# Autodesk Inventor assembly: 6 Axis Manipulator Assembly
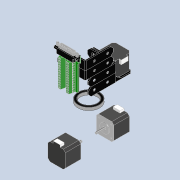
[picture p0: Inventor's stored thumbnail of the model, 180x180]
Saved by Autodesk Inventor 2022 (Build 260153000, 153)
## iProperties
Created: 2021-12-24
Part Number: 6 Axis Manipulator Assembly
Document SubType Name: Assembly
Designer: Coy
Author: Coy
## Documents named in this file (6)
- H:\3D Files\Project 3D Models\Breakfast Maker 2000\Assemblys\6 Axis Manipulator Assembly.iam
- H:\3D Files\Project 3D Models\Breakfast Maker 2000\Motors\Nema 17 Stepper Motor 37mm.ipt
- H:\3D Files\Project 3D Models\Breakfast Maker 2000\90 deg Shelf 4 Hole Bracket.ipt
- H:\3D Files\Project 3D Models\Breakfast Maker 2000\Bearings\40mm ID 52mm OD 7mm Deep Roller Bearing (2021_08_15 23_37_01 UTC).ipt
- H:\3D Files\Project 3D Models\Breakfast Maker 2000\25Pin D SUB Male Connector.ipt
- H:\3D Files\Project 3D Models\Breakfast Maker 2000\Nema 17 Stepper Motor Mounting Bracket.ipt
## Components (10 placed, 5 different names)
1. Nema 17 Stepper Motor 37mm:1
2. Nema 17 Stepper Motor 37mm:2
3. Nema 17 Stepper Motor 37mm:3 — Mate:5, Mate:6, Angle:1
4. 90 deg Shelf 4 Hole Bracket:1 — Mate:1, Flush:1, Flush:2
5. 90 deg Shelf 4 Hole Bracket:2 — Mate:1, Flush:1, Flush:2, Flush:3, Mate:3, Flush:6
6. 90 deg Shelf 4 Hole Bracket:3 — Flush:3, Flush:4, Mate:2, Flush:5, Mate:3, Flush:6, Flush:7, Flush:8
7. 90 deg Shelf 4 Hole Bracket:4 — Flush:4, Mate:2, Flush:5, Mate:4
8. 40mm ID 52mm OD 7mm Deep Roller Bearing (2021_08_15 23_37_01 UTC):1
9. 25Pin D SUB Male Connector:1
10. Nema 17 Stepper Motor Mounting Bracket:1 — Mate:4, Flush:7, Flush:8, Mate:5, Mate:6, Angle:1
## Relationships (15: Flush 8, Mate 6, Angle 1)
- Mate:1: 90 deg Shelf 4 Hole Bracket:1 ↔ 90 deg Shelf 4 Hole Bracket:2
- Flush:1: 90 deg Shelf 4 Hole Bracket:1 ↔ 90 deg Shelf 4 Hole Bracket:2
- Flush:2: 90 deg Shelf 4 Hole Bracket:1 ↔ 90 deg Shelf 4 Hole Bracket:2
- Flush:3: 90 deg Shelf 4 Hole Bracket:2 ↔ 90 deg Shelf 4 Hole Bracket:3
- Flush:4: 90 deg Shelf 4 Hole Bracket:3 ↔ 90 deg Shelf 4 Hole Bracket:4
- Mate:2: 90 deg Shelf 4 Hole Bracket:3 ↔ 90 deg Shelf 4 Hole Bracket:4
- Flush:5: 90 deg Shelf 4 Hole Bracket:3 ↔ 90 deg Shelf 4 Hole Bracket:4
- Mate:3: 90 deg Shelf 4 Hole Bracket:2 ↔ 90 deg Shelf 4 Hole Bracket:3
- Flush:6 (8.2 mm): 90 deg Shelf 4 Hole Bracket:2 ↔ 90 deg Shelf 4 Hole Bracket:3
- Mate:4: 90 deg Shelf 4 Hole Bracket:4 ↔ Nema 17 Stepper Motor Mounting Bracket:1
- Flush:7 (-2 mm): 90 deg Shelf 4 Hole Bracket:3 ↔ Nema 17 Stepper Motor Mounting Bracket:1
- Flush:8 (4.4 mm): 90 deg Shelf 4 Hole Bracket:3 ↔ Nema 17 Stepper Motor Mounting Bracket:1
- Mate:5: Nema 17 Stepper Motor 37mm:3 ↔ Nema 17 Stepper Motor Mounting Bracket:1
- Mate:6: Nema 17 Stepper Motor 37mm:3 ↔ Nema 17 Stepper Motor Mounting Bracket:1
- Angle:1 (0 deg): Nema 17 Stepper Motor 37mm:3 ↔ Nema 17 Stepper Motor Mounting Bracket:1
